# Autodesk Inventor assembly: PZT Assembly Through
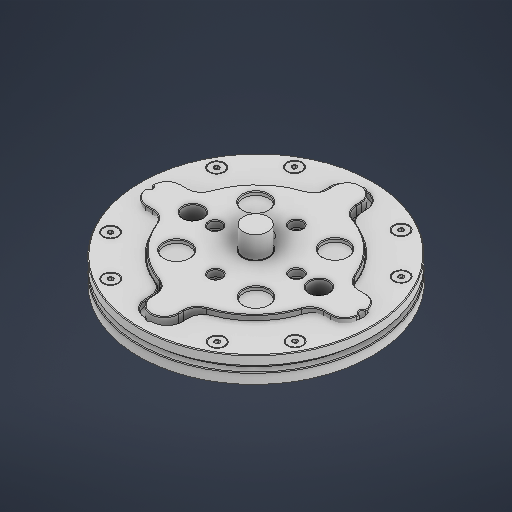
[picture p0: Inventor's stored thumbnail of the model, 512x512]
Saved by Autodesk Inventor 2025 (Build 290162000, 162)
## iProperties
Created: 2024-07-01
Part Number: PZT Assembly Through
Document SubType Name: Assembly
Designer: mayhe
Author: mayhe
## Documents named in this file (8)
- C:\Users\mayhe\OneDrive\Documents\GitHub\In-situ-monitoring-of-powder-bed-fusion-additive-manufacturing\system_development\Orichalcum\v0.2\Hardware_design\pzt-parts\PZT Assembly Through.iam
- C:\Users\mayhe\OneDrive\Documents\GitHub\In-situ-monitoring-of-powder-bed-fusion-additive-manufacturing\system_development\Orichalcum\v0.2\Hardware_design\pzt-parts\Build Plateform.ipt
- C:\Users\mayhe\OneDrive\Documents\GitHub\In-situ-monitoring-of-powder-bed-fusion-additive-manufacturing\system_development\Orichalcum\v0.2\Hardware_design\pzt-parts\Clamp Ring.ipt
- C:\Users\mayhe\OneDrive\Documents\GitHub\In-situ-monitoring-of-powder-bed-fusion-additive-manufacturing\system_development\Orichalcum\v0.2\Hardware_design\pzt-parts\91294A208_Black-Oxide Alloy Steel Hex Drive F.ipt
- C:\Users\mayhe\OneDrive\Documents\GitHub\In-situ-monitoring-of-powder-bed-fusion-additive-manufacturing\system_development\Orichalcum\v0.2\Hardware_design\pzt-parts\91290.ipt
- C:\Users\mayhe\OneDrive\Documents\GitHub\In-situ-monitoring-of-powder-bed-fusion-additive-manufacturing\system_development\Orichalcum\v0.2\Hardware_design\pzt-parts\substrate plate 12mm hole.ipt
- C:\Users\mayhe\OneDrive\Documents\GitHub\In-situ-monitoring-of-powder-bed-fusion-additive-manufacturing\system_development\Orichalcum\v0.2\Hardware_design\pzt-parts\CMG024 Transducer.ipt
- C:\Users\mayhe\OneDrive\Documents\GitHub\In-situ-monitoring-of-powder-bed-fusion-additive-manufacturing\system_development\Orichalcum\v0.2\Hardware_design\pzt-parts\Build Plateform Indents.ipt
## Components (15 placed, 7 different names)
1. Build Plateform:1 — Mate:1, Rotational:3, Rotational:18
2. Clamp Ring:1 — Mate:1, Rotational:3, Rotational:9, Rotational:10, Rotational:11, Rotational:12, Rotational:13, Rotational:14, Rotational:15, Rotational:16, Rotational:19
3. substrate plate 12mm hole:1 — Rotational:17
4. CMG024 Transducer:1 — Rotational:17, Rotational:18
5. Build Plateform Indents:1 — Rotational:19
6. 91294A208_Black-Oxide Alloy Steel Hex Drive F:1 — Rotational:9
7. 91294A208_Black-Oxide Alloy Steel Hex Drive F:2 — Rotational:10
8. 91294A208_Black-Oxide Alloy Steel Hex Drive F:3 — Rotational:11
9. 91294A208_Black-Oxide Alloy Steel Hex Drive F:4 — Rotational:12
10. 91294A208_Black-Oxide Alloy Steel Hex Drive F:5 — Rotational:15
11. 91294A208_Black-Oxide Alloy Steel Hex Drive F:6 — Rotational:16
12. 91294A208_Black-Oxide Alloy Steel Hex Drive F:7 — Rotational:13
13. 91294A208_Black-Oxide Alloy Steel Hex Drive F:8 — Rotational:14
14. 91290:1
15. 91290:2
## Relationships (13: RevoluteJoint 12, Mate 1)
- Mate:1: Build Plateform:1 ↔ Clamp Ring:1
- Rotational:3 [RevoluteJoint]: Build Plateform:1 ↔ Clamp Ring:1
- Rotational:9 [RevoluteJoint]: Clamp Ring:1 ↔ 91294A208_Black-Oxide Alloy Steel Hex Drive F:1
- Rotational:10 [RevoluteJoint]: Clamp Ring:1 ↔ 91294A208_Black-Oxide Alloy Steel Hex Drive F:2
- Rotational:11 [RevoluteJoint]: Clamp Ring:1 ↔ 91294A208_Black-Oxide Alloy Steel Hex Drive F:3
- Rotational:12 [RevoluteJoint]: Clamp Ring:1 ↔ 91294A208_Black-Oxide Alloy Steel Hex Drive F:4
- Rotational:13 [RevoluteJoint]: Clamp Ring:1 ↔ 91294A208_Black-Oxide Alloy Steel Hex Drive F:7
- Rotational:14 [RevoluteJoint]: Clamp Ring:1 ↔ 91294A208_Black-Oxide Alloy Steel Hex Drive F:8
- Rotational:15 [RevoluteJoint]: Clamp Ring:1 ↔ 91294A208_Black-Oxide Alloy Steel Hex Drive F:5
- Rotational:16 [RevoluteJoint]: Clamp Ring:1 ↔ 91294A208_Black-Oxide Alloy Steel Hex Drive F:6
- Rotational:17 [RevoluteJoint]: substrate plate 12mm hole:1 ↔ CMG024 Transducer:1
- Rotational:18 [RevoluteJoint]: Build Plateform:1 ↔ CMG024 Transducer:1
- Rotational:19 [RevoluteJoint]: Clamp Ring:1 ↔ Build Plateform Indents:1
